# Autodesk Inventor assembly: KangKang
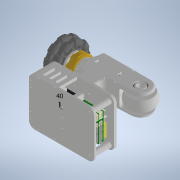
[picture p0: Inventor's stored thumbnail of the model, 180x180]
Saved by Autodesk Inventor 2020 (Build 240168000, 168)
## iProperties
Created: 2020-01-03
Part Number: KangKang
Document SubType Name: Assembly
Designer: my
Author: my
## Documents named in this file (15)
- C:\Users\my\Desktop\KangKangBalancing\KangKang.iam
- C:\Users\my\Desktop\KangKangBalancing\Turnigy 5208.ipt
- C:\Users\my\Desktop\KangKangBalancing\100mm-Plastic-Omni-Wheel.iam
- C:\Users\my\Desktop\KangKangBalancing\omniwheel_mount.ipt
- C:\Users\my\Desktop\KangKangBalancing\bodyL.ipt
- C:\Users\my\Desktop\KangKangBalancing\battery2500.ipt
- C:\Users\my\Desktop\KangKangBalancing\tarot_5008_340kv\tarot_5008_340kv_assy.iam
- C:\Users\my\Desktop\KangKangBalancing\Body-R.ipt
- C:\Users\my\Desktop\KangKangBalancing\fleet.ipt
- C:\Users\my\Desktop\KangKangBalancing\front wheelnewVer.ipt
- C:\Users\my\Desktop\KangKangBalancing\fleet_top.ipt
- C:\Users\my\Desktop\KangKangBalancing\mjvesc_v0.1\MJVESC_v01.iam
- C:\Users\my\Desktop\KangKangBalancing\bearing25x32x4.ipt
- C:\Users\my\Desktop\KangKangBalancing\AS5147_3D_Export\Inventor_AS5147_ENC_ANGLE_VER01\AS5147_ENC_ANGLE_VER01.iam
- C:\Users\my\Desktop\KangKangBalancing\AS5147_3D_Export\Inventor_AS5147_VERTICAL_ANGLE_VER01\AS5147_ENC_VERTICAL_VER01.iam
## Components (15 placed, 14 different names)
1. Turnigy 5208:1 — Mate:1, Mate:2, Mate:5, Mate:6, Mate:9, Mate:36
2. 100mm-Plastic-Omni-Wheel:1 [sub-assembly] — Mate:1, Mate:4
3. omniwheel_mount:1 — Mate:2, Mate:4, Mate:36
4. bodyL:1 — Mate:5, Mate:6, Mate:9, Mate:10, Mate:11, Mate:12, Mate:15, Mate:16, Mate:17, Mate:18, Flush:1, Mate:23, Mate:24, Flush:2, Flush:3, Mate:33, Mate:34, Mate:35, Mate:37, Mate:38, Mate:39, Mate:40, Mate:41, Mate:42
5. battery2500:1 — Mate:17, Mate:18, Mate:23
6. tarot_5008_340kv_assy:1 [sub-assembly] — Mate:10, Mate:11, Mate:12, Mate:25, Mate:26
7. Body-R:1 — Mate:15, Mate:16, Flush:1
8. fleet:1 — Mate:24, Flush:2, Flush:3, Mate:27, Mate:28, Flush:4, Mate:30, Flush:7, Flush:8
9. front wheelnewVer:1 — Mate:25, Mate:26, Mate:31, Mate:32
10. fleet_top:1 — Mate:27, Mate:28, Flush:4
11. MJVESC_v01:1 [sub-assembly] — Flush:5, Flush:6, Mate:29, Mate:30, Flush:8
12. MJVESC_v01:2 [sub-assembly] — Flush:5, Flush:6, Mate:29, Flush:7
13. bearing25x32x4:1 — Mate:31, Mate:32
14. AS5147_ENC_ANGLE_VER01:1 [sub-assembly] — Mate:37, Mate:38, Mate:39
15. AS5147_ENC_VERTICAL_VER01:1 [sub-assembly] — Mate:40, Mate:41, Mate:42
## Relationships (41: Mate 33, Flush 8)
- Mate:1: Turnigy 5208:1 ↔ 100mm-Plastic-Omni-Wheel:1
- Mate:2: Turnigy 5208:1 ↔ omniwheel_mount:1
- Mate:4: 100mm-Plastic-Omni-Wheel:1 ↔ omniwheel_mount:1
- Mate:5: Turnigy 5208:1 ↔ bodyL:1
- Mate:6: Turnigy 5208:1 ↔ bodyL:1
- Mate:9: Turnigy 5208:1 ↔ bodyL:1
- Mate:10: bodyL:1 ↔ tarot_5008_340kv_assy:1
- Mate:11: bodyL:1 ↔ tarot_5008_340kv_assy:1
- Mate:12: bodyL:1 ↔ tarot_5008_340kv_assy:1
- Mate:15: bodyL:1 ↔ Body-R:1
- Mate:16: bodyL:1 ↔ Body-R:1
- Mate:17 (1.5 mm): bodyL:1 ↔ battery2500:1
- Mate:18 (1 mm): bodyL:1 ↔ battery2500:1
- Flush:1: bodyL:1 ↔ Body-R:1
- Mate:23: bodyL:1 ↔ battery2500:1
- Mate:24: bodyL:1 ↔ fleet:1
- Flush:2: bodyL:1 ↔ fleet:1
- Flush:3: bodyL:1 ↔ fleet:1
- Mate:25: tarot_5008_340kv_assy:1 ↔ front wheelnewVer:1
- Mate:26: tarot_5008_340kv_assy:1 ↔ front wheelnewVer:1
- Mate:27: fleet:1 ↔ fleet_top:1
- Mate:28: fleet:1 ↔ fleet_top:1
- Flush:4: fleet:1 ↔ fleet_top:1
- Flush:5: MJVESC_v01:1 ↔ MJVESC_v01:2
- Flush:6: MJVESC_v01:1 ↔ MJVESC_v01:2
- Mate:29: MJVESC_v01:1 ↔ MJVESC_v01:2
- Mate:30 (12 mm): fleet:1 ↔ MJVESC_v01:1
- Flush:7 (25 mm): fleet:1 ↔ MJVESC_v01:2
- Flush:8 (18 mm): fleet:1 ↔ MJVESC_v01:1
- Mate:31: front wheelnewVer:1 ↔ bearing25x32x4:1
- Mate:32: front wheelnewVer:1 ↔ bearing25x32x4:1
- Mate:33: bodyL:1
- Mate:34: bodyL:1
- Mate:35: bodyL:1
- Mate:36: Turnigy 5208:1 ↔ omniwheel_mount:1
- Mate:37: bodyL:1 ↔ AS5147_ENC_ANGLE_VER01:1
- Mate:38: bodyL:1 ↔ AS5147_ENC_ANGLE_VER01:1
- Mate:39: bodyL:1 ↔ AS5147_ENC_ANGLE_VER01:1
- Mate:40: bodyL:1 ↔ AS5147_ENC_VERTICAL_VER01:1
- Mate:41: bodyL:1 ↔ AS5147_ENC_VERTICAL_VER01:1
- Mate:42: bodyL:1 ↔ AS5147_ENC_VERTICAL_VER01:1
